# Autodesk Inventor assembly: Table
(part 2 of 2)
- メイト:231 [Mate]: SFK-N19T:9 ↔ JIS B 1176 - メートル M8 x 12:59
- メイト:232 [Mate]: SFK-N19T:9 ↔ JIS B 1176 - メートル M8 x 12:59
- メイト:233 [Mate]: SFK-N19T:9 ↔ JIS B 1176 - メートル M8 x 12:60
- メイト:234 [Mate]: SFK-N19T:9 ↔ JIS B 1176 - メートル M8 x 12:60
- メイト:235 [Mate]: SFK-N19T:32 ↔ JIS B 1176 - メートル M8 x 12:61
- メイト:236 [Mate]: SFK-N19T:32 ↔ JIS B 1176 - メートル M8 x 12:61
- メイト:237 [Mate]: SFK-N19T:32 ↔ JIS B 1176 - メートル M8 x 12:62
- メイト:238 [Mate]: SFK-N19T:32 ↔ JIS B 1176 - メートル M8 x 12:62
- メイト:239 [Mate]: SFK-N19T:2 ↔ JIS B 1176 - メートル M8 x 12:63
- メイト:240 [Mate]: SFK-N19T:2 ↔ JIS B 1176 - メートル M8 x 12:63
- メイト:241 [Mate]: SFK-N19T:2 ↔ JIS B 1176 - メートル M8 x 12:64
- メイト:242 [Mate]: SFK-N19T:2 ↔ JIS B 1176 - メートル M8 x 12:64
- メイト:243 [Mate]: SFK-N19T:6 ↔ JIS B 1176 - メートル M8 x 12:65
- メイト:244 [Mate]: SFK-N19T:6 ↔ JIS B 1176 - メートル M8 x 12:65
- メイト:245 [Mate]: SFK-N19T:6 ↔ JIS B 1176 - メートル M8 x 12:66
- メイト:246 [Mate]: SFK-N19T:6 ↔ JIS B 1176 - メートル M8 x 12:66
- 挿入:15 [Insert]: SFK-N19T:2 ↔ JIS B 1176 - メートル M8 x 12:67
- 挿入:16 [Insert]: SFK-N19T:2 ↔ JIS B 1176 - メートル M8 x 12:68
- 挿入:17 [Insert]: SFK-N19T:23 ↔ JIS B 1176 - メートル M8 x 12:69
- 挿入:18 [Insert]: SFK-N19T:23 ↔ JIS B 1176 - メートル M8 x 12:70
- メイト:247 [Mate]: SFK-N19T:25 ↔ JIS B 1176 - メートル M8 x 12:71
- メイト:248 [Mate]: SFK-N19T:25 ↔ JIS B 1176 - メートル M8 x 12:71
- メイト:249 [Mate]: SFK-N19T:25 ↔ JIS B 1176 - メートル M8 x 12:72
- メイト:250 [Mate]: SFK-N19T:25 ↔ JIS B 1176 - メートル M8 x 12:72
- 挿入:19 [Insert]: SFK-N19T:5 ↔ JIS B 1176 - メートル M8 x 12:73
- 挿入:20 [Insert]: SFK-N19T:5 ↔ JIS B 1176 - メートル M8 x 12:74
- 挿入:21 [Insert]: SFK-N19T:32 ↔ JIS B 1176 - メートル M8 x 12:75
- 挿入:22 [Insert]: SFK-N19T:32 ↔ JIS B 1176 - メートル M8 x 12:76
- メイト:251 [Mate]: SFK-N19T:35 ↔ JIS B 1176 - メートル M8 x 12:77
- メイト:252 [Mate]: SFK-N19T:35 ↔ JIS B 1176 - メートル M8 x 12:77
- メイト:253 [Mate]: SFK-N19T:35 ↔ JIS B 1176 - メートル M8 x 12:78
- メイト:254 [Mate]: SFK-N19T:35 ↔ JIS B 1176 - メートル M8 x 12:78
- 挿入:23 [Insert]: SFK-N19T:6 ↔ JIS B 1176 - メートル M8 x 12:79
- 挿入:24 [Insert]: SFK-N19T:6 ↔ JIS B 1176 - メートル M8 x 12:80
- メイト:255 [Mate]: SFK-N19T:9 ↔ JIS B 1176 - メートル M8 x 12:81
- メイト:256 [Mate]: SFK-N19T:9 ↔ JIS B 1176 - メートル M8 x 12:81
- メイト:257 [Mate]: SFK-N19T:9 ↔ JIS B 1176 - メートル M8 x 12:82
- メイト:258 [Mate]: SFK-N19T:9 ↔ JIS B 1176 - メートル M8 x 12:82
- メイト:259 [Mate]: SFK-N19T:24 ↔ JIS B 1176 - メートル M8 x 12:83
- メイト:260 [Mate]: SFK-N19T:24 ↔ JIS B 1176 - メートル M8 x 12:83
- メイト:261 [Mate]: SFK-N19T:24 ↔ JIS B 1176 - メートル M8 x 12:84
- メイト:262 [Mate]: SFK-N19T:24 ↔ JIS B 1176 - メートル M8 x 12:84
- 挿入:25 [Insert]: SFK-N19T:24 ↔ JIS B 1176 - メートル M8 x 12:85
- 挿入:26 [Insert]: SFK-N19T:24 ↔ JIS B 1176 - メートル M8 x 12:86
- メイト:263 [Mate]: SFK-N19T:21 ↔ JIS B 1176 - メートル M8 x 12:87
- メイト:264 [Mate]: SFK-N19T:21 ↔ JIS B 1176 - メートル M8 x 12:87
- メイト:265 [Mate]: SFK-N19T:21 ↔ JIS B 1176 - メートル M8 x 12:88
- メイト:266 [Mate]: SFK-N19T:21 ↔ JIS B 1176 - メートル M8 x 12:88
- メイト:267 [Mate]: SFK-N19T:23 ↔ JIS B 1176 - メートル M8 x 12:89
- メイト:268 [Mate]: SFK-N19T:23 ↔ JIS B 1176 - メートル M8 x 12:89
- メイト:269 [Mate]: SFK-N19T:23 ↔ JIS B 1176 - メートル M8 x 12:90
- メイト:270 [Mate]: SFK-N19T:23 ↔ JIS B 1176 - メートル M8 x 12:90
- 挿入:27 [Insert]: SFK-N19T:50 ↔ JIS B 1176 - メートル M8 x 12:91
- 挿入:28 [Insert]: SFK-N19T:50 ↔ JIS B 1176 - メートル M8 x 12:92
- 挿入:29 [Insert]: SFK-N19T:30 ↔ JIS B 1176 - メートル M8 x 12:93
- 挿入:30 [Insert]: SFK-N19T:30 ↔ JIS B 1176 - メートル M8 x 12:94
- 挿入:31 [Insert]: SFK-N19T:45 ↔ JIS B 1176 - メートル M8 x 12:95
- 挿入:32 [Insert]: SFK-N19T:45 ↔ JIS B 1176 - メートル M8 x 12:96
- 挿入:33 [Insert]: SFK-N19T:29 ↔ JIS B 1176 - メートル M8 x 12:97
- 挿入:34 [Insert]: SFK-N19T:29 ↔ JIS B 1176 - メートル M8 x 12:98
- メイト:271 [Mate]: SFK-N19T:38 ↔ JIS B 1176 - メートル M8 x 12:99
- メイト:272 [Mate]: SFK-N19T:38 ↔ JIS B 1176 - メートル M8 x 12:99
- メイト:273 [Mate]: SFK-N19T:38 ↔ JIS B 1176 - メートル M8 x 12:100
- メイト:274 [Mate]: SFK-N19T:38 ↔ JIS B 1176 - メートル M8 x 12:100
- メイト:275 [Mate]: SFK-N19T:13 ↔ JIS B 1176 - メートル M8 x 12:101
- メイト:276 [Mate]: SFK-N19T:13 ↔ JIS B 1176 - メートル M8 x 12:101
- メイト:277 [Mate]: SFK-N19T:13 ↔ JIS B 1176 - メートル M8 x 12:102
- メイト:278 [Mate]: SFK-N19T:13 ↔ JIS B 1176 - メートル M8 x 12:102
- 挿入:35 [Insert]: SFK-N19T:49 ↔ JIS B 1176 - メートル M8 x 12:103
- 挿入:36 [Insert]: SFK-N19T:49 ↔ JIS B 1176 - メートル M8 x 12:104
- 挿入:37 [Insert]: SFK-N19T:14 ↔ JIS B 1176 - メートル M8 x 12:105
- 挿入:38 [Insert]: SFK-N19T:14 ↔ JIS B 1176 - メートル M8 x 12:106
- 挿入:39 [Insert]: SFK-N19T:46 ↔ JIS B 1176 - メートル M8 x 12:107
- 挿入:40 [Insert]: SFK-N19T:46 ↔ JIS B 1176 - メートル M8 x 12:108
- 挿入:41 [Insert]: SFK-N19T:46 ↔ JIS B 1176 - メートル M8 x 12:109
- 挿入:42 [Insert]: SFK-N19T:46 ↔ JIS B 1176 - メートル M8 x 12:110
- 挿入:43 [Insert]: SFK-N19T:47 ↔ JIS B 1176 - メートル M8 x 12:111
- 挿入:44 [Insert]: SFK-N19T:47 ↔ JIS B 1176 - メートル M8 x 12:112
- 挿入:45 [Insert]: SFK-N19T:8 ↔ JIS B 1176 - メートル M8 x 12:113
- 挿入:46 [Insert]: SFK-N19T:8 ↔ JIS B 1176 - メートル M8 x 12:114
- 挿入:47 [Insert]: SFK-N19T:49 ↔ JIS B 1176 - メートル M8 x 12:115
- 挿入:48 [Insert]: SFK-N19T:49 ↔ JIS B 1176 - メートル M8 x 12:116
- 挿入:49 [Insert]: SFK-N19T:40 ↔ JIS B 1176 - メートル M8 x 12:117
- 挿入:50 [Insert]: SFK-N19T:40 ↔ JIS B 1176 - メートル M8 x 12:118
- 挿入:51 [Insert]: SFK-N19T:40 ↔ JIS B 1176 - メートル M8 x 12:119
- 挿入:52 [Insert]: SFK-N19T:40 ↔ JIS B 1176 - メートル M8 x 12:120
- 挿入:53 [Insert]: SFK-N19T:56 ↔ JIS B 1176 - メートル M8 x 12:121
- 挿入:54 [Insert]: SFK-N19T:56 ↔ JIS B 1176 - メートル M8 x 12:122
- 挿入:55 [Insert]: SFK-N19T:8 ↔ JIS B 1176 - メートル M8 x 12:123
- 挿入:56 [Insert]: SFK-N19T:8 ↔ JIS B 1176 - メートル M8 x 12:124
- 挿入:57 [Insert]: SFK-N19T:14 ↔ JIS B 1176 - メートル M8 x 12:125
- 挿入:58 [Insert]: SFK-N19T:14 ↔ JIS B 1176 - メートル M8 x 12:126
- 挿入:59 [Insert]: SFK-N19T:18 ↔ JIS B 1176 - メートル M8 x 12:127
- 挿入:60 [Insert]: SFK-N19T:18 ↔ JIS B 1176 - メートル M8 x 12:128
- 挿入:61 [Insert]: SFK-N19T:18 ↔ JIS B 1176 - メートル M8 x 12:129
- 挿入:62 [Insert]: SFK-N19T:18 ↔ JIS B 1176 - メートル M8 x 12:130
- 挿入:63 [Insert]: SFK-N19T:51 ↔ JIS B 1176 - メートル M8 x 12:131
- 挿入:64 [Insert]: SFK-N19T:51 ↔ JIS B 1176 - メートル M8 x 12:132
- 挿入:65 [Insert]: SFK-N19T:47 ↔ JIS B 1176 - メートル M8 x 12:133
- 挿入:66 [Insert]: SFK-N19T:47 ↔ JIS B 1176 - メートル M8 x 12:134
- 挿入:67 [Insert]: SFK-N19T:16 ↔ JIS B 1176 - メートル M8 x 12:135
- 挿入:68 [Insert]: SFK-N19T:16 ↔ JIS B 1176 - メートル M8 x 12:136
- 挿入:69 [Insert]: SFK-N19T:39 ↔ JIS B 1176 - メートル M8 x 12:137
- 挿入:70 [Insert]: SFK-N19T:39 ↔ JIS B 1176 - メートル M8 x 12:138
- 挿入:71 [Insert]: SFK-N19T:39 ↔ JIS B 1176 - メートル M8 x 12:139
- 挿入:72 [Insert]: SFK-N19T:39 ↔ JIS B 1176 - メートル M8 x 12:140
- 挿入:73 [Insert]: SFK-N19T:52 ↔ JIS B 1176 - メートル M8 x 12:141
- 挿入:74 [Insert]: SFK-N19T:52 ↔ JIS B 1176 - メートル M8 x 12:142
- メイト:279 [Mate]: SFK-N19T:51 ↔ JIS B 1176 - メートル M8 x 12:143
- メイト:280 [Mate]: SFK-N19T:51 ↔ JIS B 1176 - メートル M8 x 12:143
- メイト:281 [Mate]: SFK-N19T:51 ↔ JIS B 1176 - メートル M8 x 12:144
- メイト:282 [Mate]: SFK-N19T:51 ↔ JIS B 1176 - メートル M8 x 12:144
- 挿入:75 [Insert]: SFK-N19T:16 ↔ JIS B 1176 - メートル M8 x 12:145
- 挿入:76 [Insert]: SFK-N19T:16 ↔ JIS B 1176 - メートル M8 x 12:146
- メイト:283 [Mate]: SFK-N19T:55 ↔ JIS B 1176 - メートル M8 x 12:147
- メイト:284 [Mate]: SFK-N19T:55 ↔ JIS B 1176 - メートル M8 x 12:147
- メイト:285 [Mate]: SFK-N19T:55 ↔ JIS B 1176 - メートル M8 x 12:148
- メイト:286 [Mate]: SFK-N19T:55 ↔ JIS B 1176 - メートル M8 x 12:148
- 挿入:77 [Insert]: SFK-N19T:17 ↔ JIS B 1176 - メートル M8 x 12:149
- 挿入:78 [Insert]: SFK-N19T:17 ↔ JIS B 1176 - メートル M8 x 12:150
- 挿入:79 [Insert]: SFK-N19T:3 ↔ JIS B 1176 - メートル M8 x 12:151
- 挿入:80 [Insert]: SFK-N19T:3 ↔ JIS B 1176 - メートル M8 x 12:152
- 挿入:81 [Insert]: SFK-N19T:20 ↔ JIS B 1176 - メートル M8 x 12:153
- 挿入:82 [Insert]: SFK-N19T:20 ↔ JIS B 1176 - メートル M8 x 12:154
- 挿入:83 [Insert]: SFK-N19T:37 ↔ JIS B 1176 - メートル M8 x 12:155
- 挿入:84 [Insert]: SFK-N19T:37 ↔ JIS B 1176 - メートル M8 x 12:156
- 挿入:85 [Insert]: SFK-N19T:53 ↔ JIS B 1176 - メートル M8 x 12:157
- 挿入:86 [Insert]: SFK-N19T:53 ↔ JIS B 1176 - メートル M8 x 12:158
- 挿入:87 [Insert]: SFK-N19T:20 ↔ JIS B 1176 - メートル M8 x 12:159
- 挿入:88 [Insert]: SFK-N19T:20 ↔ JIS B 1176 - メートル M8 x 12:160
- メイト:287 [Mate]: SFK-N19T:15 ↔ JIS B 1176 - メートル M8 x 12:161
- メイト:288 [Mate]: SFK-N19T:15 ↔ JIS B 1176 - メートル M8 x 12:161
- メイト:289 [Mate]: SFK-N19T:15 ↔ JIS B 1176 - メートル M8 x 12:162
- メイト:290 [Mate]: SFK-N19T:15 ↔ JIS B 1176 - メートル M8 x 12:162
- メイト:291 [Mate]: SFK-N19T:10 ↔ JIS B 1176 - メートル M8 x 12:163
- メイト:292 [Mate]: SFK-N19T:10 ↔ JIS B 1176 - メートル M8 x 12:163
- メイト:293 [Mate]: SFK-N19T:10 ↔ JIS B 1176 - メートル M8 x 12:164
- メイト:294 [Mate]: SFK-N19T:10 ↔ JIS B 1176 - メートル M8 x 12:164
- 挿入:89 [Insert]: SFK-N19T:17 ↔ JIS B 1176 - メートル M8 x 12:165
- 挿入:90 [Insert]: SFK-N19T:17 ↔ JIS B 1176 - メートル M8 x 12:166
- 挿入:91 [Insert]: SFK-N19T:31 ↔ JIS B 1176 - メートル M8 x 12:167
- 挿入:92 [Insert]: SFK-N19T:31 ↔ JIS B 1176 - メートル M8 x 12:168
- 挿入:93 [Insert]: SFK-N19T:31 ↔ JIS B 1176 - メートル M8 x 12:169
- 挿入:94 [Insert]: SFK-N19T:31 ↔ JIS B 1176 - メートル M8 x 12:170
- 挿入:95 [Insert]: SFK-N19T:37 ↔ JIS B 1176 - メートル M8 x 12:171
- 挿入:96 [Insert]: SFK-N19T:37 ↔ JIS B 1176 - メートル M8 x 12:172
- 挿入:97 [Insert]: SFK-N19T:28 ↔ JIS B 1176 - メートル M8 x 12:173
- 挿入:98 [Insert]: SFK-N19T:28 ↔ JIS B 1176 - メートル M8 x 12:174
- 挿入:99 [Insert]: SFK-N19T:27 ↔ JIS B 1176 - メートル M8 x 12:175
- 挿入:100 [Insert]: SFK-N19T:27 ↔ JIS B 1176 - メートル M8 x 12:176
- メイト:295 [Mate]: SFK-N19T:22 ↔ JIS B 1176 - メートル M8 x 12:177
- メイト:296 [Mate]: SFK-N19T:22 ↔ JIS B 1176 - メートル M8 x 12:177
- メイト:297 [Mate]: SFK-N19T:22 ↔ JIS B 1176 - メートル M8 x 12:178
- メイト:298 [Mate]: SFK-N19T:22 ↔ JIS B 1176 - メートル M8 x 12:178
- 挿入:101 [Insert]: SFK-N19T:28 ↔ JIS B 1176 - メートル M8 x 12:179
- 挿入:102 [Insert]: SFK-N19T:28 ↔ JIS B 1176 - メートル M8 x 12:180
- 挿入:103 [Insert]: SFK-N19T:15 ↔ JIS B 1176 - メートル M8 x 12:181
- 挿入:104 [Insert]: SFK-N19T:15 ↔ JIS B 1176 - メートル M8 x 12:182
- 挿入:105 [Insert]: SFK-N19T:48 ↔ JIS B 1176 - メートル M8 x 12:183
- 挿入:106 [Insert]: SFK-N19T:48 ↔ JIS B 1176 - メートル M8 x 12:184
- 挿入:107 [Insert]: SFK-N19T:48 ↔ JIS B 1176 - メートル M8 x 12:185
- 挿入:108 [Insert]: SFK-N19T:48 ↔ JIS B 1176 - メートル M8 x 12:186
- メイト:299 [Mate]: SFK-N19T:53 ↔ JIS B 1176 - メートル M8 x 12:187
- メイト:300 [Mate]: SFK-N19T:53 ↔ JIS B 1176 - メートル M8 x 12:187
- メイト:301 [Mate]: SFK-N19T:53 ↔ JIS B 1176 - メートル M8 x 12:188
- メイト:302 [Mate]: SFK-N19T:53 ↔ JIS B 1176 - メートル M8 x 12:188
- 挿入:109 [Insert]: SFK-N19T:55 ↔ JIS B 1176 - メートル M8 x 12:189
- 挿入:110 [Insert]: SFK-N19T:55 ↔ JIS B 1176 - メートル M8 x 12:190
- 挿入:111 [Insert]: SFK-N19T:52 ↔ JIS B 1176 - メートル M8 x 12:191
- 挿入:112 [Insert]: SFK-N19T:52 ↔ JIS B 1176 - メートル M8 x 12:192
- 挿入:113 [Insert]: SFK-N19T:12 ↔ JIS B 1176 - メートル M8 x 12:193
- 挿入:114 [Insert]: SFK-N19T:12 ↔ JIS B 1176 - メートル M8 x 12:194
- メイト:303 [Mate]: SFK-N19T:3 ↔ JIS B 1176 - メートル M8 x 12:195
- メイト:304 [Mate]: SFK-N19T:3 ↔ JIS B 1176 - メートル M8 x 12:195
- メイト:305 [Mate]: SFK-N19T:3 ↔ JIS B 1176 - メートル M8 x 12:196
- メイト:306 [Mate]: SFK-N19T:3 ↔ JIS B 1176 - メートル M8 x 12:196
- 挿入:115 [Insert]: SFK-N19T:10 ↔ JIS B 1176 - メートル M8 x 12:197
- 挿入:116 [Insert]: SFK-N19T:10 ↔ JIS B 1176 - メートル M8 x 12:198
- 挿入:117 [Insert]: SFK-N19T:27 ↔ JIS B 1176 - メートル M8 x 12:199
- 挿入:118 [Insert]: SFK-N19T:27 ↔ JIS B 1176 - メートル M8 x 12:200
- 挿入:119 [Insert]: SFK-N19T:44 ↔ JIS B 1176 - メートル M8 x 12:201
- 挿入:120 [Insert]: SFK-N19T:44 ↔ JIS B 1176 - メートル M8 x 12:202
- 挿入:121 [Insert]: SFK-N19T:50 ↔ JIS B 1176 - メートル M8 x 12:203
- 挿入:122 [Insert]: SFK-N19T:50 ↔ JIS B 1176 - メートル M8 x 12:204
- 挿入:123 [Insert]: SFK-N19T:22 ↔ JIS B 1176 - メートル M8 x 12:205
- 挿入:124 [Insert]: SFK-N19T:22 ↔ JIS B 1176 - メートル M8 x 12:206
- メイト:307 [Mate]: EFS8-4040-1100:2 ↔ board:1
- フラッシュ:113 [Flush]: EFS8-4040-1100:3 ↔ board:1
- フラッシュ:114 [Flush]: EFS8-4040-580:1 ↔ board:1
- 挿入:125 [Insert]: board:1 ↔ JIS B 1176 - メートル M6 x 10:1
- 挿入:126 [Insert]: board:1 ↔ JIS B 1176 - メートル M6 x 10:2
- 挿入:127 [Insert]: board:1 ↔ JIS B 1176 - メートル M6 x 10:3
- 挿入:128 [Insert]: board:1 ↔ JIS B 1176 - メートル M6 x 10:4
- 挿入:129 [Insert]: board:1 ↔ JIS B 1176 - メートル M6 x 10:5
- 挿入:130 [Insert]: board:1 ↔ JIS B 1176 - メートル M6 x 10:6
- 挿入:131 [Insert]: board:1 ↔ JIS B 1176 - メートル M6 x 10:7
- 挿入:132 [Insert]: board:1 ↔ JIS B 1176 - メートル M6 x 10:8
- 挿入:133 [Insert]: board:1 ↔ JIS B 1176 - メートル M6 x 10:9
- 挿入:134 [Insert]: board:1 ↔ JIS B 1176 - メートル M6 x 10:10
- 挿入:135 [Insert]: board:1 ↔ JIS B 1176 - メートル M6 x 10:11
- 挿入:136 [Insert]: board:1 ↔ JIS B 1176 - メートル M6 x 10:12
- 挿入:137 [Insert]: board:1 ↔ JIS B 1176 - メートル M6 x 10:13
- 挿入:138 [Insert]: board:1 ↔ JIS B 1176 - メートル M6 x 10:14
- 挿入:139 [Insert]: board:1 ↔ JIS B 1176 - メートル M6 x 10:15
- 挿入:140 [Insert]: board:1 ↔ JIS B 1176 - メートル M6 x 10:16
- 挿入:141 [Insert]: board:1 ↔ JIS B 1176 - メートル M6 x 10:17
- 挿入:142 [Insert]: board:1 ↔ JIS B 1176 - メートル M6 x 10:18
- 挿入:143 [Insert]: board:1 ↔ JIS B 1176 - メートル M6 x 10:19
- 挿入:144 [Insert]: board:1 ↔ JIS B 1176 - メートル M6 x 10:20
- 挿入:145 [Insert]: board:1 ↔ JIS B 1176 - メートル M6 x 10:21
- 挿入:146 [Insert]: board:1 ↔ JIS B 1176 - メートル M6 x 10:22
- フラッシュ:115 [Flush]: EFS8-4040-1100:4 ↔ foot_parts:1
- フラッシュ:116 [Flush]: EFS8-4040-580:6 ↔ foot_parts:1
- メイト:308 [Mate]: EFS8-4040-580:6 ↔ foot_parts:1
- フラッシュ:117 [Flush]: EFS8-4040-1100:1 ↔ foot_parts:2
- フラッシュ:118 [Flush]: EFS8-4040-580:6 ↔ foot_parts:2
- メイト:309 [Mate]: EFS8-4040-580:6 ↔ foot_parts:2
- フラッシュ:119 [Flush]: EFS8-4040-580:2 ↔ foot_parts:3
- フラッシュ:120 [Flush]: EFS8-4040-1100:1 ↔ foot_parts:3
- メイト:310 [Mate]: EFS8-4040-1100:1 ↔ foot_parts:3
- フラッシュ:121 [Flush]: EFS8-4040-1100:4 ↔ foot_parts:4
- フラッシュ:122 [Flush]: EFS8-4040-580:2 ↔ foot_parts:4
- メイト:311 [Mate]: EFS8-4040-1100:4 ↔ foot_parts:4
- メイト:312 [Mate] (-550 mm): board:1
- フラッシュ:123 [Flush]: board:1
- メイト:313 [Mate] (-330 mm): EFS8-4040-1100:3
